# Autodesk Inventor assembly: Stopa v3
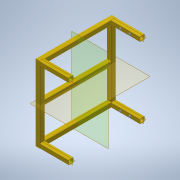
[picture p0: Inventor's stored thumbnail of the model, 180x180]
Saved by Autodesk Inventor 2021 (Build 250183000, 183)
## iProperties
Created: 2024-04-18
Part Number: Stopa v3
Document SubType Name: Assembly
Designer: Michal
Author: Michal
## Documents named in this file (5)
- C:\Users\Michal\Documents\GitHub\PNW_PhotoBoothFrame_3D\Stopa v3.iam
- C:\Users\Michal\Documents\GitHub\PNW_PhotoBoothFrame_3D\Stopa v1 profil 1.ipt
- C:\Users\Michal\Documents\GitHub\PNW_PhotoBoothFrame_3D\Stopa v1 profil 2.ipt
- C:\Users\Michal\Documents\GitHub\PNW_PhotoBoothFrame_3D\Stopa v1 profil 3.ipt
- C:\Users\Michal\Documents\GitHub\PNW_PhotoBoothFrame_3D\M8x15.ipt
## Components (17 placed, 4 different names)
1. Stopa v1 profil 1:1 — Mate:1, Flush:1, Mate:2, Mate:5, Mate:6, Mate:8, Mate:10, Mate:26, Mate:27, Flush:10, Mate:33
2. Stopa v1 profil 1:2 — Mate:1, Flush:1, Mate:2, Flush:2, Mate:3, Mate:7, Flush:4, Mate:28, Mate:31, Mate:32
3. Stopa v1 profil 1:3 — Flush:2, Flush:3, Mate:3, Mate:4, Mate:29, Mate:30, Flush:11
4. Stopa v1 profil 1:4 — Flush:3, Mate:4, Mate:5, Mate:6, Mate:9, Mate:34, Mate:35
5. Stopa v1 profil 2:1 — Mate:7, Flush:4, Mate:11, Mate:12
6. Stopa v1 profil 3:1 — Mate:12, Mate:14, Mate:15, Mate:16, Mate:26, Mate:33, Mate:34
7. M8x15:1 — Mate:14, Flush:6, Mate:16
8. M8x15:2 — Mate:15, Flush:6
9. Stopa v1 profil 3:2 — Mate:27, Flush:10, Mate:32
10. M8x15:3
11. M8x15:4
12. Stopa v1 profil 3:3 — Mate:28, Mate:30, Mate:31
13. M8x15:5
14. M8x15:6
15. Stopa v1 profil 3:4 — Mate:29, Mate:35, Flush:11
16. M8x15:7
17. M8x15:8
## Relationships (44: Mate 34, Flush 10)
- Mate:1: Stopa v1 profil 1:1 ↔ Stopa v1 profil 1:2
- Flush:1: Stopa v1 profil 1:1 ↔ Stopa v1 profil 1:2
- Mate:2: Stopa v1 profil 1:1 ↔ Stopa v1 profil 1:2
- Flush:2: Stopa v1 profil 1:2 ↔ Stopa v1 profil 1:3
- Flush:3: Stopa v1 profil 1:3 ↔ Stopa v1 profil 1:4
- Mate:3: Stopa v1 profil 1:2 ↔ Stopa v1 profil 1:3
- Mate:4: Stopa v1 profil 1:3 ↔ Stopa v1 profil 1:4
- Mate:5: Stopa v1 profil 1:1 ↔ Stopa v1 profil 1:4
- Mate:6: Stopa v1 profil 1:1 ↔ Stopa v1 profil 1:4
- Mate:7: Stopa v1 profil 1:2 ↔ Stopa v1 profil 2:1
- Flush:4: Stopa v1 profil 1:2 ↔ Stopa v1 profil 2:1
- Mate:8: Stopa v1 profil 1:1
- Mate:9: Stopa v1 profil 1:4
- Mate:10: Stopa v1 profil 1:1
- Mate:11: Stopa v1 profil 2:1
- Mate:12: Stopa v1 profil 2:1 ↔ Stopa v1 profil 3:1
- Mate:14: Stopa v1 profil 3:1 ↔ M8x15:1
- Mate:15: Stopa v1 profil 3:1 ↔ M8x15:2
- Flush:6: M8x15:1 ↔ M8x15:2
- Mate:16 (3 mm): Stopa v1 profil 3:1 ↔ M8x15:1
- [Mate]: Stopa v1 profil 3:2 ↔ M8x15:3
- [Mate]: Stopa v1 profil 3:2 ↔ M8x15:4
- [Flush]: M8x15:3 ↔ M8x15:4
- [Mate] (3 mm): Stopa v1 profil 3:2 ↔ M8x15:3
- [Mate]: Stopa v1 profil 3:3 ↔ M8x15:5
- [Mate]: Stopa v1 profil 3:3 ↔ M8x15:6
- [Flush]: M8x15:5 ↔ M8x15:6
- [Mate] (3 mm): Stopa v1 profil 3:3 ↔ M8x15:5
- [Mate]: Stopa v1 profil 3:4 ↔ M8x15:7
- [Mate]: Stopa v1 profil 3:4 ↔ M8x15:8
- [Flush]: M8x15:7 ↔ M8x15:8
- [Mate] (3 mm): Stopa v1 profil 3:4 ↔ M8x15:7
- Mate:26: Stopa v1 profil 1:1 ↔ Stopa v1 profil 3:1
- Mate:27: Stopa v1 profil 1:1 ↔ Stopa v1 profil 3:2
- Mate:28: Stopa v1 profil 1:2 ↔ Stopa v1 profil 3:3
- Mate:29: Stopa v1 profil 1:3 ↔ Stopa v1 profil 3:4
- Mate:30: Stopa v1 profil 1:3 ↔ Stopa v1 profil 3:3
- Mate:31: Stopa v1 profil 1:2 ↔ Stopa v1 profil 3:3
- Flush:10: Stopa v1 profil 1:1 ↔ Stopa v1 profil 3:2
- Mate:32: Stopa v1 profil 1:2 ↔ Stopa v1 profil 3:2
- Mate:33: Stopa v1 profil 1:1 ↔ Stopa v1 profil 3:1
- Mate:34: Stopa v1 profil 1:4 ↔ Stopa v1 profil 3:1
- Mate:35: Stopa v1 profil 1:4 ↔ Stopa v1 profil 3:4
- Flush:11: Stopa v1 profil 1:3 ↔ Stopa v1 profil 3:4
## Named parameters: d32_d28 = 0 mm, d33_d29 = 0 mm, d34_d30 = 0 mm, d35_d31 = 3 mm, d36_d28 = 0 mm, d37_d29 = 0 mm, d38_d30 = 0 mm, d39_d31 = 3 mm, d40_d28 = 0 mm, d41_d29 = 0 mm, d42_d30 = 0 mm, d43_d31 = 3 mm
